# Autodesk Inventor assembly: Clock Board V2
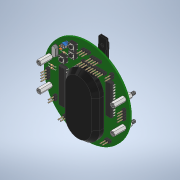
[picture p0: Inventor's stored thumbnail of the model, 180x180]
Saved by Autodesk Inventor 2020 (Build 240168000, 168)
## iProperties
Company: A Company
Created: 2019-07-06
Part Number: Clock Board V2
Description: KiCad electronic assembly
Document SubType Name: Assembly
Designer: andwh
Authority: Unknown
Sending System: KiCad to STEP converter
Preprocessor: Open CASCADE STEP processor 6.9
Title: Clock Board V2.step
Author: An Author
## Documents named in this file (17)
- C:\Users\andwh\Documents\Projects\Clock Clock\PCB\Clock Board V2\Clock Board V2.iam
- C:\Users\andwh\Documents\Projects\Clock Clock\PCB\Clock Board V2\PinHeader_1x06_P2.54mm_Vertical.iam
- C:\Users\andwh\Documents\Projects\Clock Clock\PCB\Clock Board V2\PinHeader_1x03_P2.54mm_Vertical.iam
- C:\Users\andwh\Documents\Projects\Clock Clock\PCB\Clock Board V2\PinHeader_1x02_P2.54mm_Vertical.iam
- C:\Users\andwh\Documents\Projects\Clock Clock\PCB\Clock Board V2\R_Axial_DIN0204_L3.6mm_D1.6mm_P7.62mm_Horizontal.iam
- C:\Users\andwh\Documents\Projects\Clock Clock\PCB\Clock Board V2\C_Disc_D3.0mm_W1.6mm_P2.50mm.iam
- C:\Users\andwh\Documents\Projects\Clock Clock\PCB\Clock Board V2\Crystal_HC49-U_Vertical.iam
- C:\Users\andwh\Documents\Projects\Clock Clock\PCB\Clock Board V2\CP_Radial_D5.0mm_P2.50mm.iam
- C:\Users\andwh\Documents\Projects\Clock Clock\PCB\Clock Board V2\DIP-24_W7.62mm.iam
- C:\Users\andwh\Documents\Projects\Clock Clock\PCB\Clock Board V2\DIP-28_W7.62mm.iam
- C:\Users\andwh\Documents\Projects\Clock Clock\PCB\Clock Board V2\SW_PUSH_6mm.iam
- C:\Users\andwh\Documents\Projects\Clock Clock\PCB\Clock Board V2\COMPOUND.ipt
- C:\Users\andwh\Documents\Projects\Clock Clock\Parts\BKA30D-R5.ipt
- C:\Users\andwh\Documents\Projects\Clock Clock\Parts\95783A051_NYLON 6-6 MALE-FEM THRDED HEX STANDOFF.ipt
- C:\Users\andwh\Documents\Projects\Clock Clock\Parts\95783A059_NYLON 6-6 MALE-FEM THRDED HEX STANDOFF.ipt
- C:\Users\andwh\Documents\Projects\Clock Clock\CC-bottomHand.ipt
- C:\Users\andwh\Documents\Projects\Clock Clock\CC-topHand.ipt
## Components (37 placed, 31 different names)
1. 2 [sub-assembly]
2. 4 [sub-assembly]
3. 5 [sub-assembly]
4. 7 [sub-assembly]
5. 8 [sub-assembly]
6. 9 [sub-assembly]
7. 10 [sub-assembly]
8. 11 [sub-assembly]
9. 12 [sub-assembly]
10. 13 [sub-assembly]
11. 14 [sub-assembly]
12. 15 [sub-assembly]
13. 16 [sub-assembly]
14. 18 [sub-assembly]
15. 19 [sub-assembly]
16. 20 [sub-assembly]
17. 22 [sub-assembly]
18. 23 [sub-assembly]
19. 25 [sub-assembly]
20. 27 [sub-assembly]
21. 29 [sub-assembly]
22. 31 [sub-assembly]
23. 33 [sub-assembly]
24. 34 [sub-assembly]
25. 35 [sub-assembly]
26. 36 — Insert:1, Insert:2, Insert:3, Insert:4
27. BKA30D-R5:1 — Insert:1, Insert:2, Insert:5, Insert:6
28. CC-bottomHand:1 — Insert:5
29. CC-topHand:1 — Insert:6
30. 95783A059_NYLON 6-6 MALE-FEM THRDED HEX STANDOFF:1 — Insert:3
31. 95783A051_NYLON 6-6 MALE-FEM THRDED HEX STANDOFF:1 — Insert:4
32. 95783A059_NYLON 6-6 MALE-FEM THRDED HEX STANDOFF:2
33. 95783A051_NYLON 6-6 MALE-FEM THRDED HEX STANDOFF:2
34. 95783A059_NYLON 6-6 MALE-FEM THRDED HEX STANDOFF:3
35. 95783A051_NYLON 6-6 MALE-FEM THRDED HEX STANDOFF:3
36. 95783A059_NYLON 6-6 MALE-FEM THRDED HEX STANDOFF:4
37. 95783A051_NYLON 6-6 MALE-FEM THRDED HEX STANDOFF:4
## Component patterns: (4 elements, first: 95783A059_NYLON 6-6 MALE-FEM THRDED HEX STANDOFF:1 + 95783A051_NYLON 6-6 MALE-FEM THRDED HEX STANDOFF:1)
## Relationships (6: Insert 6)
- Insert:1: 36 ↔ BKA30D-R5:1
- Insert:2: 36 ↔ BKA30D-R5:1
- Insert:3: 36 ↔ 95783A059_NYLON 6-6 MALE-FEM THRDED HEX STANDOFF:1
- Insert:4: 36 ↔ 95783A051_NYLON 6-6 MALE-FEM THRDED HEX STANDOFF:1
- Insert:5: BKA30D-R5:1 ↔ CC-bottomHand:1
- Insert:6: BKA30D-R5:1 ↔ CC-topHand:1
